# Autodesk Inventor assembly: Assembly
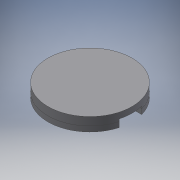
[picture p0: Inventor's stored thumbnail of the model, 180x180]
Saved by Autodesk Inventor 2018 (Build 220112000, 112)
## iProperties
Created: 2017-07-21
Part Number: Assembly
Document SubType Name: Assembly
Designer: Micha
Author: Micha
## Documents named in this file (4)
- C:\Users\Micha\Documents\Coding_Projects\Wifi_Pixels\3D\Assembly.iam
- C:\Users\Micha\Documents\Coding_Projects\Wifi_Pixels\3D\Bottom_v1.ipt
- C:\Users\Micha\Documents\Coding_Projects\Wifi_Pixels\3D\Diffuser_V1.ipt
- C:\Users\Micha\Documents\Coding_Projects\Wifi_Pixels\3D\WifiPixels.ipt
## Components (3 placed, 3 different names)
1. Bottom_v1:1 — Mate:1, Insert:1, Flush:1, Insert:2, Insert:3
2. Diffuser_V1:1 — Mate:1, Insert:1, Flush:1
3. WifiPixels:1 — Insert:2, Insert:3
## Relationships (5: Insert 3, Mate 1, Flush 1)
- Mate:1: Bottom_v1:1 ↔ Diffuser_V1:1
- Insert:1: Bottom_v1:1 ↔ Diffuser_V1:1
- Flush:1: Bottom_v1:1 ↔ Diffuser_V1:1
- Insert:2: Bottom_v1:1 ↔ WifiPixels:1
- Insert:3: Bottom_v1:1 ↔ WifiPixels:1
